# Autodesk Inventor assembly: Left Hook Encoder Assembly
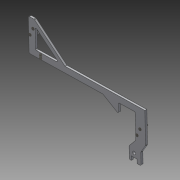
[picture p0: Inventor's stored thumbnail of the model, 180x180]
Saved by Autodesk Inventor 2014 SP1 (Build 180222100, 222)
## iProperties
Created: 2013-03-16
Part Number: Left Hook Encoder Assembly
Document SubType Name: Assembly
Designer: Arpan
Mass: 288.368 g
Surface Area: 498.509 cm^2
Volume: 109.48 cm^3
Density: 2.63398 g/cm^3
Author: Arpan
## Documents named in this file (6)
- C:\Users\Moses\Documents\Inventor\Sally Rebuild\Rebuild Sally\Left Hook Encoder Assembly.iam
- C:\Users\Moses\Documents\Inventor\Sally Rebuild\Rebuild Sally\7779K630.ipt
- C:\Users\Moses\Documents\Inventor\Sally Rebuild\Rebuild Sally\Rebuild Left Climber Hook.ipt
- C:\Users\Moses\Documents\Inventor\Sally Rebuild\Rebuild Sally\4-40 18-8 Stainless Steel Pan Head Phillips Machine Screw\18-8 Stainless Steel Machine Screw Hex Nut\91841A005.ipt
- C:\Users\Moses\Documents\Inventor\Sally Rebuild\Rebuild Sally\4-40 18-8 Stainless Steel Pan Head Phillips Machine Screw\1.0000\91772A115.ipt
- C:\Users\Moses\Documents\Inventor\Sally Rebuild\Rebuild Sally\Standard #4 Washer.ipt
## Components (17 placed, 5 different names)
1. Rebuild Left Climber Hook:1 — Mate:1, Mate:2, Mate:3, Mate:4, Mate:5, Mate:6, Insert:5, Insert:6, Insert:7, Insert:8, Insert:9, Insert:10
2. 7779K630:1 — Mate:2, Mate:3, Mate:4, Insert:1, Insert:2
3. 7779K630:2 — Mate:1, Mate:5, Mate:6, Insert:3, Insert:4
4. 91841A005:1 — Insert:1
5. 91841A005:2 — Insert:2
6. 91841A005:3 — Insert:3
7. 91841A005:4 — Insert:4
8. 91772A115:1 — Insert:11
9. 91772A115:2 — Insert:12
10. 91772A115:3 — Insert:13
11. 91772A115:4 — Insert:14
12. Standard #4 Washer:1 — Insert:5, Insert:11
13. Standard #4 Washer:2 — Insert:6, Insert:12
14. Standard #4 Washer:3 — Insert:7
15. Standard #4 Washer:4 — Insert:8
16. Standard #4 Washer:5 — Insert:9, Insert:13
17. Standard #4 Washer:6 — Insert:10, Insert:14
## Relationships (20: Insert 14, Mate 6)
- Mate:1: Rebuild Left Climber Hook:1 ↔ 7779K630:2
- Mate:2: Rebuild Left Climber Hook:1 ↔ 7779K630:1
- Mate:3: Rebuild Left Climber Hook:1 ↔ 7779K630:1
- Mate:4: Rebuild Left Climber Hook:1 ↔ 7779K630:1
- Mate:5: Rebuild Left Climber Hook:1 ↔ 7779K630:2
- Mate:6: Rebuild Left Climber Hook:1 ↔ 7779K630:2
- Insert:1: 7779K630:1 ↔ 91841A005:1
- Insert:2: 7779K630:1 ↔ 91841A005:2
- Insert:3: 7779K630:2 ↔ 91841A005:3
- Insert:4: 7779K630:2 ↔ 91841A005:4
- Insert:5: Rebuild Left Climber Hook:1 ↔ Standard #4 Washer:1
- Insert:6: Rebuild Left Climber Hook:1 ↔ Standard #4 Washer:2
- Insert:7: Rebuild Left Climber Hook:1 ↔ Standard #4 Washer:3
- Insert:8: Rebuild Left Climber Hook:1 ↔ Standard #4 Washer:4
- Insert:9: Rebuild Left Climber Hook:1 ↔ Standard #4 Washer:5
- Insert:10: Rebuild Left Climber Hook:1 ↔ Standard #4 Washer:6
- Insert:11: 91772A115:1 ↔ Standard #4 Washer:1
- Insert:12: 91772A115:2 ↔ Standard #4 Washer:2
- Insert:13: 91772A115:3 ↔ Standard #4 Washer:5
- Insert:14: 91772A115:4 ↔ Standard #4 Washer:6
